# Autodesk Inventor assembly: ASSY,MK4i,Swerve_Module,HIGH
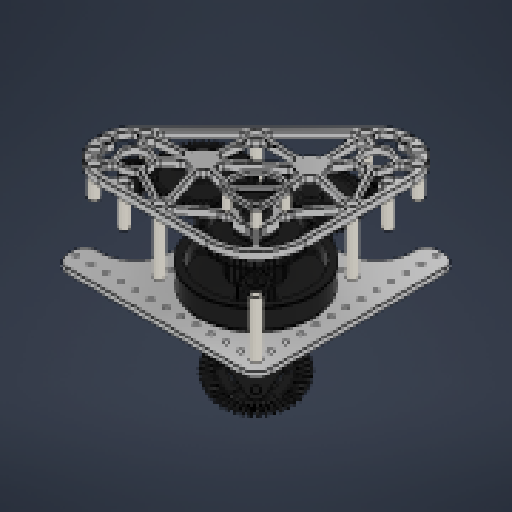
[picture p0: Inventor's stored thumbnail of the model, 512x512]
Saved by Autodesk Inventor 2026.1 (Build 301233020, 233B)
## iProperties
Created: 2024-01-10
Part Number: ASSY,MK4i,Swerve_Module,HIGH
Document SubType Name: Assembly
Designer: dave.simone
Mass: 1631.73 g
Surface Area: 2686.09 cm^2
Volume: 361.803 cm^3
Density: 4.51 g/cm^3
Author: dave.simone
## Documents named in this file (8)
- C:\Users\Owen\Documents\GitHub\2026-Robot-Mechanical\#1_CAD Library\SDS MK4i Swerve\ASSY,MK4i,HIGH,Swerve_Module.iam
- C:\Users\Owen\Documents\GitHub\2026-Robot-Mechanical\#1_CAD Library\SDS MK4i Swerve\PURCHASED_SUB,PLATE,MAIN,MK4i,Swerve.ipt
- C:\Users\Owen\Documents\GitHub\2026-Robot-Mechanical\#1_CAD Library\SDS MK4i Swerve\PURCHASED_SUB,PLATE,UPPER,MK4i,Swerve.ipt
- C:\Users\Owen\Documents\GitHub\2026-Robot-Mechanical\#1_CAD Library\SDS MK4i Swerve\PURCHASED_SUB,PLATE,ENCODER,MK4i,Swerve.ipt
- C:\Users\Owen\Documents\GitHub\2026-Robot-Mechanical\#1_CAD Library\SDS MK4i Swerve\PURCHASED_SUB,SPACER,SHORT,MK4i,Swerve.ipt
- C:\Users\Owen\Documents\GitHub\2026-Robot-Mechanical\#1_CAD Library\SDS MK4i Swerve\PURCHASED_SUB,SPACER,LONG,MK4i,Swerve.ipt
- C:\Users\Owen\Documents\GitHub\2026-Robot-Mechanical\#1_CAD Library\SDS MK4i Swerve\PURCHASED_SUB,SPACER,SHORTER,MK4i,Swerve.ipt
- C:\Users\Owen\Documents\GitHub\2026-Robot-Mechanical\#1_CAD Library\SDS MK4i Swerve\PURCHASED_SUB,GEAR_TRAIN,WHEEL,MK4i,Swerve.ipt
## Components (17 placed, 7 different names)
1. PURCHASED_SUB,GEAR_TRAIN,WHEEL,MK4i,Swerve:1 — Mate:20, Mate:21
2. PURCHASED_SUB,PLATE,MAIN,MK4i,Swerve:1 — Mate:6, Mate:7, Mate:8, Mate:9, Insert:13, Mate:20, Mate:21
3. PURCHASED_SUB,PLATE,UPPER,MK4i,Swerve:1 — Insert:4, Insert:5, Insert:6, Insert:7, Insert:8, Insert:9, Insert:10, Insert:11, Insert:12, Insert:20, Insert:21, Insert:22
4. PURCHASED_SUB,SPACER,SHORTER,MK4i,Swerve:1 — Insert:20, Mate:11
5. PURCHASED_SUB,SPACER,SHORTER,MK4i,Swerve:2 — Insert:21, Mate:12
6. PURCHASED_SUB,SPACER,SHORTER,MK4i,Swerve:3 — Insert:22, Mate:13
7. PURCHASED_SUB,SPACER,LONG,MK4i,Swerve:4 — Insert:13
8. PURCHASED_SUB,PLATE,ENCODER,MK4i,Swerve:1 — Mate:11, Mate:12, Mate:13
9. PURCHASED_SUB,SPACER,LONG,MK4i,Swerve:1 — Insert:4, Mate:6, Mate:7
10. PURCHASED_SUB,SPACER,LONG,MK4i,Swerve:2 — Insert:5, Mate:8
11. PURCHASED_SUB,SPACER,LONG,MK4i,Swerve:3 — Insert:6, Mate:9
12. PURCHASED_SUB,SPACER,SHORT,MK4i,Swerve:4 — Insert:8
13. PURCHASED_SUB,SPACER,SHORT,MK4i,Swerve:5 — Insert:7
14. PURCHASED_SUB,SPACER,SHORT,MK4i,Swerve:6 — Insert:9
15. PURCHASED_SUB,SPACER,SHORT,MK4i,Swerve:7 — Insert:10
16. PURCHASED_SUB,SPACER,SHORT,MK4i,Swerve:8 — Insert:11
17. PURCHASED_SUB,SPACER,SHORT,MK4i,Swerve:9 — Insert:12
## Relationships (22: Insert 13, Mate 9)
- Insert:4: PURCHASED_SUB,PLATE,UPPER,MK4i,Swerve:1 ↔ PURCHASED_SUB,SPACER,LONG,MK4i,Swerve:1
- Insert:5: PURCHASED_SUB,PLATE,UPPER,MK4i,Swerve:1 ↔ PURCHASED_SUB,SPACER,LONG,MK4i,Swerve:2
- Insert:6: PURCHASED_SUB,PLATE,UPPER,MK4i,Swerve:1 ↔ PURCHASED_SUB,SPACER,LONG,MK4i,Swerve:3
- Mate:6: PURCHASED_SUB,PLATE,MAIN,MK4i,Swerve:1 ↔ PURCHASED_SUB,SPACER,LONG,MK4i,Swerve:1
- Mate:7: PURCHASED_SUB,PLATE,MAIN,MK4i,Swerve:1 ↔ PURCHASED_SUB,SPACER,LONG,MK4i,Swerve:1
- Mate:8: PURCHASED_SUB,PLATE,MAIN,MK4i,Swerve:1 ↔ PURCHASED_SUB,SPACER,LONG,MK4i,Swerve:2
- Mate:9: PURCHASED_SUB,PLATE,MAIN,MK4i,Swerve:1 ↔ PURCHASED_SUB,SPACER,LONG,MK4i,Swerve:3
- Insert:7: PURCHASED_SUB,PLATE,UPPER,MK4i,Swerve:1 ↔ PURCHASED_SUB,SPACER,SHORT,MK4i,Swerve:5
- Insert:8: PURCHASED_SUB,PLATE,UPPER,MK4i,Swerve:1 ↔ PURCHASED_SUB,SPACER,SHORT,MK4i,Swerve:4
- Insert:9: PURCHASED_SUB,PLATE,UPPER,MK4i,Swerve:1 ↔ PURCHASED_SUB,SPACER,SHORT,MK4i,Swerve:6
- Insert:10: PURCHASED_SUB,PLATE,UPPER,MK4i,Swerve:1 ↔ PURCHASED_SUB,SPACER,SHORT,MK4i,Swerve:7
- Insert:11: PURCHASED_SUB,PLATE,UPPER,MK4i,Swerve:1 ↔ PURCHASED_SUB,SPACER,SHORT,MK4i,Swerve:8
- Insert:12: PURCHASED_SUB,PLATE,UPPER,MK4i,Swerve:1 ↔ PURCHASED_SUB,SPACER,SHORT,MK4i,Swerve:9
- Insert:13: PURCHASED_SUB,PLATE,MAIN,MK4i,Swerve:1 ↔ PURCHASED_SUB,SPACER,LONG,MK4i,Swerve:4
- Insert:20: PURCHASED_SUB,PLATE,UPPER,MK4i,Swerve:1 ↔ PURCHASED_SUB,SPACER,SHORTER,MK4i,Swerve:1
- Insert:21: PURCHASED_SUB,PLATE,UPPER,MK4i,Swerve:1 ↔ PURCHASED_SUB,SPACER,SHORTER,MK4i,Swerve:2
- Insert:22: PURCHASED_SUB,PLATE,UPPER,MK4i,Swerve:1 ↔ PURCHASED_SUB,SPACER,SHORTER,MK4i,Swerve:3
- Mate:11: PURCHASED_SUB,SPACER,SHORTER,MK4i,Swerve:1 ↔ PURCHASED_SUB,PLATE,ENCODER,MK4i,Swerve:1
- Mate:12: PURCHASED_SUB,SPACER,SHORTER,MK4i,Swerve:2 ↔ PURCHASED_SUB,PLATE,ENCODER,MK4i,Swerve:1
- Mate:13: PURCHASED_SUB,SPACER,SHORTER,MK4i,Swerve:3 ↔ PURCHASED_SUB,PLATE,ENCODER,MK4i,Swerve:1
- Mate:20: PURCHASED_SUB,GEAR_TRAIN,WHEEL,MK4i,Swerve:1 ↔ PURCHASED_SUB,PLATE,MAIN,MK4i,Swerve:1
- Mate:21: PURCHASED_SUB,GEAR_TRAIN,WHEEL,MK4i,Swerve:1 ↔ PURCHASED_SUB,PLATE,MAIN,MK4i,Swerve:1
